# Autodesk Inventor assembly: ПД Модуль 200х140х75
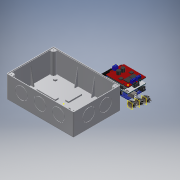
[picture p0: Inventor's stored thumbnail of the model, 180x180]
Saved by Autodesk Inventor 2019 (Build 230136000, 136)
## iProperties
Created: 2020-05-19
Part Number: ПД Модуль 200х140х75
Material: Типовые
Document SubType Name: Assembly
Designer: Surflay
Author: Surflay
## Documents named in this file (7)
- C:\Users\Surflay\Desktop\Университет\ПД\Модели\Дистанционная связь (модуль)\ПД Модуль 200х140х75.iam
- C:\Users\Surflay\Desktop\Университет\ПД\Модели\Дистанционная связь (модуль)\ПД Коробка 200х140х75.ipt
- C:\Users\Surflay\Desktop\Университет\ПД\Модели\Дистанционная связь (модуль)\A_Arduino_Uno_Wifi_Shield.iam
- C:\Users\Surflay\Desktop\Университет\ПД\Модели\Дистанционная связь (модуль)\Monster_motor_Shield.ipt
- Troyka_Shield.ipt
- C:\Users\Surflay\Desktop\Университет\ПД\Модели\Дистанционная связь (модуль)\3-pin\3-pin.iam
- C:\Users\Surflay\Desktop\Университет\ПД\Модели\Arduino MEGA 2560 R3.ipt
## Components (7 placed, 5 different names)
1. ПД Коробка 200х140х75:1 — Угол:2, Угол:3
2. Arduino MEGA 2560 R3:1 — Угол:4, Угол:5, Вставка:2
3. A_Arduino_Uno_Wifi_Shield:1 [sub-assembly] — Вставка:1, Угол:1, Угол:2, Угол:3, Угол:4, Угол:5, Вставка:2
4. Troyka_Shield:1 — Вставка:1, Угол:1
5. kls15-225-m12:1 [sub-assembly]
6. kls15-225-m12:2 [sub-assembly]
7. kls15-225-m12:3 [sub-assembly]
## Relationships (7: Angle 5, Insert 2)
- Вставка:1 [Insert] (-16 mm): A_Arduino_Uno_Wifi_Shield:1 ↔ Troyka_Shield:1
- Угол:1 [Angle] (90 deg): A_Arduino_Uno_Wifi_Shield:1 ↔ Troyka_Shield:1
- Угол:2 [Angle] (0 deg): ПД Коробка 200х140х75:1 ↔ A_Arduino_Uno_Wifi_Shield:1
- Угол:3 [Angle] (0 deg): ПД Коробка 200х140х75:1 ↔ A_Arduino_Uno_Wifi_Shield:1
- Угол:4 [Angle] (0 deg): Arduino MEGA 2560 R3:1 ↔ A_Arduino_Uno_Wifi_Shield:1
- Угол:5 [Angle] (90 deg): Arduino MEGA 2560 R3:1 ↔ A_Arduino_Uno_Wifi_Shield:1
- Вставка:2 [Insert] (-16 mm): Arduino MEGA 2560 R3:1 ↔ A_Arduino_Uno_Wifi_Shield:1
